# Autodesk Inventor assembly: Frame1
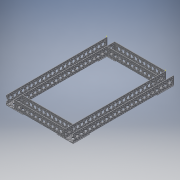
[picture p0: Inventor's stored thumbnail of the model, 180x180]
Saved by Autodesk Inventor 2016 (Build 200138000, 138)
## iProperties
Created: 2015-10-28
Part Number: Frame1
Document SubType Name: Assembly
Designer: RoboticsUser
Author: RoboticsUser
## Documents named in this file (4)
- C:\Robotics\2015-16 CAD\custom cad parts\Frame1.iam
- C:\Robotics\2015-16 CAD\COTSParts\Actobotics\585 parts\585450.ipt
- C:\Robotics\2015-16 CAD\COTSParts\Actobotics\585 parts\585466.ipt
- C:\Robotics\2015-16 CAD\COTSParts\Actobotics\585 parts\585628.ipt
## Components (8 placed, 3 different names)
1. 585450:1 — Mate:1, Flush:1, Flush:2, Mate:2, Flush:3, Flush:4, Flush:11, Flush:13
2. 585450:2 — Mate:3, Flush:5, Flush:6, Flush:10
3. 585466:1 — Mate:1, Flush:1, Flush:2, Mate:3, Flush:5, Mate:4, Flush:7, Flush:8, Mate:7, Flush:14
4. 585466:2 — Mate:2, Flush:3, Flush:4, Flush:6, Mate:5, Flush:9, Mate:6, Flush:12
5. 585628:1 — Mate:4, Flush:7, Flush:8
6. 585628:3 — Mate:6, Flush:11, Flush:12
7. 585628:4 — Mate:7, Flush:13, Flush:14
8. 585628:5 — Mate:5, Flush:9, Flush:10
## Relationships (21: Flush 14, Mate 7)
- Mate:1: 585450:1 ↔ 585466:1
- Flush:1: 585450:1 ↔ 585466:1
- Flush:2: 585450:1 ↔ 585466:1
- Mate:2: 585450:1 ↔ 585466:2
- Flush:3: 585450:1 ↔ 585466:2
- Flush:4: 585450:1 ↔ 585466:2
- Mate:3: 585450:2 ↔ 585466:1
- Flush:5: 585450:2 ↔ 585466:1
- Flush:6: 585450:2 ↔ 585466:2
- Mate:4: 585466:1 ↔ 585628:1
- Flush:7: 585466:1 ↔ 585628:1
- Flush:8: 585466:1 ↔ 585628:1
- Mate:5: 585466:2 ↔ 585628:5
- Flush:9: 585466:2 ↔ 585628:5
- Flush:10: 585450:2 ↔ 585628:5
- Mate:6: 585466:2 ↔ 585628:3
- Flush:11: 585450:1 ↔ 585628:3
- Flush:12: 585466:2 ↔ 585628:3
- Mate:7: 585466:1 ↔ 585628:4
- Flush:13: 585450:1 ↔ 585628:4
- Flush:14: 585466:1 ↔ 585628:4
